# Autodesk Inventor assembly: Gantry
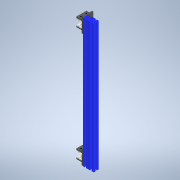
[picture p0: Inventor's stored thumbnail of the model, 180x180]
Saved by Autodesk Inventor 2022.3 (Build 263350000, 350)
## iProperties
Created: 2022-04-08
Part Number: Gantry
Document SubType Name: Assembly
Designer: Robert Nies
Author: Robert Nies
## Documents named in this file (3)
- C:\Users\rober\PycharmProjects\CNCRouter\Master Assembly\Gantry\Gantry.iam
- C:\Users\rober\PycharmProjects\CNCRouter\Stock Parts\Linear Motion\Linear Bearing.iam
- C:\Users\rober\PycharmProjects\CNCRouter\Master Assembly\Gantry\Gantry Cross Beam.ipt
## Components (3 placed, 2 different names)
1. Linear Bearing:1 [sub-assembly] — Flush:1, Flush:2, Mate:1
2. Linear Bearing:2 [sub-assembly] — Flush:1, Flush:2, Mate:1, Mate:2, Flush:3, Flush:4
3. Gantry Cross Beam:1 — Mate:2, Flush:3, Flush:4
## Relationships (6: Flush 4, Mate 2)
- Flush:1: Linear Bearing:1 ↔ Linear Bearing:2
- Flush:2: Linear Bearing:1 ↔ Linear Bearing:2
- Mate:1 (-762 mm): Linear Bearing:1 ↔ Linear Bearing:2
- Mate:2: Linear Bearing:2 ↔ Gantry Cross Beam:1
- Flush:3: Linear Bearing:2 ↔ Gantry Cross Beam:1
- Flush:4 (-2.54 mm): Linear Bearing:2 ↔ Gantry Cross Beam:1
